# Autodesk Inventor assembly: Assembly1
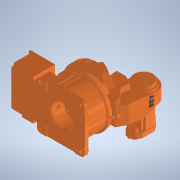
[picture p0: Inventor's stored thumbnail of the model, 180x180]
Saved by Autodesk Inventor 2021 (Build 250183000, 183)
## iProperties
Created: 2020-12-06
Part Number: Assembly1
Document SubType Name: Assembly
Designer: juanj
Author: juanj
## Documents named in this file (3)
- C:\Users\juanj\OneDrive - Universidad Politécnica de Madrid\Máster\Primer semestre\Diseño y control de robots\REPOSITORIO\Robot-ABB\Assembly1.iam
- C:\Users\juanj\OneDrive - Universidad Politécnica de Madrid\Máster\Primer semestre\Diseño y control de robots\REPOSITORIO\Robot-ABB\Base.ipt
- C:\Users\juanj\OneDrive - Universidad Politécnica de Madrid\Máster\Primer semestre\Diseño y control de robots\REPOSITORIO\Robot-ABB\Link1.ipt
## Components (2 placed, 2 different names)
1. Base — Insert:1
2. Link1 — Insert:1
## Relationships (1: Insert 1)
- Insert:1: Base ↔ Link1
